# Autodesk Inventor assembly: baseAndCapForSvBonyPlosse-40mm
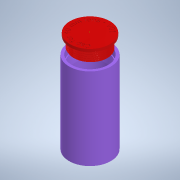
[picture p0: Inventor's stored thumbnail of the model, 180x180]
Saved by Autodesk Inventor 2021.1 (Build 251245010, 245A)
## iProperties
Created: 2020-10-09
Part Number: baseAndCapForSvBonyPlosse-40mm
Document SubType Name: Assembly
Designer: robst
Author: robst
## Documents named in this file (3)
- C:\git\CAD-Development\robSteele\ShapeWays\TelescopeProjects\eyepieceCases\baseAndCapForSvBonyPlosse-40mm.iam
- C:\git\CAD-Development\robSteele\ShapeWays\TelescopeProjects\eyepieceCases\BaseForSvBonyPlosse-40mm.ipt
- C:\git\CAD-Development\robSteele\ShapeWays\TelescopeProjects\eyepieceCases\CapForSvBonyPlosse-40mm.ipt
## Components (2 placed, 2 different names)
1. BaseForSvBonyPlosse-40mm:1 — Insert:1
2. CapForSvBonyPlosse-40mm:1 — Insert:1
## Relationships (1: Insert 1)
- Insert:1 (19.05 mm): BaseForSvBonyPlosse-40mm:1 ↔ CapForSvBonyPlosse-40mm:1
